# Autodesk Inventor assembly: car
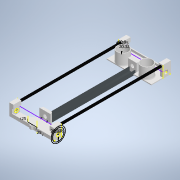
[picture p0: Inventor's stored thumbnail of the model, 180x180]
Saved by Autodesk Inventor 2020.1 (Build 241239000, 239)
## iProperties
Created: 2020-03-02
Part Number: car
Document SubType Name: Assembly
Designer: akend
Author: akend
## Documents named in this file (5)
- D:\statesCar\car.iam
- D:\statesCar\carbonnFiber.ipt
- D:\statesCar\front 3-1.ipt
- D:\statesCar\rear 3-1.ipt
- D:\statesCar\alCchannel.ipt
## Components (5 placed, 4 different names)
1. carbonnFiber:1 — Rotational:1, Rotational:2, Rigid:1, Insert:1
2. front 3-1:1 — Rotational:1, Rotational:3
3. rear 3-1:1 — Rotational:2, Rigid:1, Insert:1
4. carbonnFiber:2 — Rotational:3
5. alCchannel:1
## Relationships (5: RevoluteJoint 3, WeldJoint 1, Insert 1)
- Rotational:1 [RevoluteJoint]: carbonnFiber:1 ↔ front 3-1:1
- Rotational:2 [RevoluteJoint]: carbonnFiber:1 ↔ rear 3-1:1
- Rigid:1 [WeldJoint]: carbonnFiber:1 ↔ rear 3-1:1
- Insert:1: carbonnFiber:1 ↔ rear 3-1:1
- Rotational:3 [RevoluteJoint]: front 3-1:1 ↔ carbonnFiber:2
